# Autodesk Inventor assembly: Crankshaft assembly
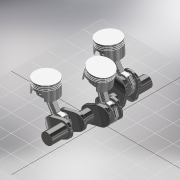
[picture p0: Inventor's stored thumbnail of the model, 180x180]
Saved by Autodesk Inventor 2019 (Build 230136000, 136)
## iProperties
Created: 2020-05-30
Part Number: Crankshaft assembly
Document SubType Name: Assembly
Designer: Manoj
Author: Manoj
## Documents named in this file (3)
- F:\Softwares\Autodesk\YOUTUBE\TotUMentors\Crankshaft assembly.iam
- F:\Softwares\Autodesk\YOUTUBE\TotUMentors\piston_assembled.iam
- F:\Softwares\Autodesk\YOUTUBE\TotUMentors\Crankshaft.ipt
## Components (4 placed, 2 different names)
1. piston_assembled:1 [sub-assembly] — Mate:3, Mate:6
2. piston_assembled:2 [sub-assembly] — Mate:1, Mate:5, Mate:7
3. piston_assembled:3 [sub-assembly] — Mate:2, Mate:4
4. Crankshaft:1 — Mate:1, Mate:2, Mate:3, Mate:4, Mate:5, Mate:6, Mate:7
## Relationships (7: Mate 7)
- Mate:1: piston_assembled:2 ↔ Crankshaft:1
- Mate:2: piston_assembled:3 ↔ Crankshaft:1
- Mate:3: piston_assembled:1 ↔ Crankshaft:1
- Mate:4 (15.24 mm): piston_assembled:3 ↔ Crankshaft:1
- Mate:5 (15.24 mm): piston_assembled:2 ↔ Crankshaft:1
- Mate:6 (15.24 mm): piston_assembled:1 ↔ Crankshaft:1
- Mate:7: piston_assembled:2 ↔ Crankshaft:1
